# Autodesk Inventor assembly: LEG2
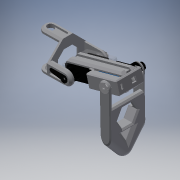
[picture p0: Inventor's stored thumbnail of the model, 180x180]
Saved by Autodesk Inventor 2017 (Build 210142000, 142)
## iProperties
Created: 2017-09-24
Part Number: LEG2
Document SubType Name: Assembly
Designer: Alexander Miller
Author: Alexander Miller
## Documents named in this file (12)
- X:\Alex\Documents\Git\HeRo-Mini\Hardware\LEG.iam
- X:\Alex\Documents\Git\HeRo-Mini\Hardware\SERVO.iam
- X:\Alex\Documents\Git\HeRo-Mini\Hardware\COXA.ipt
- X:\Alex\Documents\Git\HeRo-Mini\Hardware\FEMUR_A.ipt
- X:\Alex\Documents\Git\HeRo-Mini\Hardware\FEMUR_B.ipt
- X:\Alex\Documents\Git\HeRo-Mini\Hardware\BEARING.ipt
- X:\Alex\Documents\Git\HeRo-Mini\Hardware\TIBIA.ipt
- X:\Alex\Documents\Git\HeRo-Mini\Hardware\NUT_3MM.ipt
- X:\Alex\Documents\Git\HeRo-Mini\Hardware\NUT_2MM.ipt
- X:\Alex\Documents\Git\HeRo-Mini\Hardware\M2_SCREW_8MM.ipt
- X:\Alex\Documents\Git\HeRo-Mini\Hardware\M3_WASHER.ipt
- X:\Alex\Documents\Git\HeRo-Mini\Hardware\M3_SCREW_8MM.ipt
## Components (23 placed, 11 different names)
1. SERVO:1 [sub-assembly] — Rigid:1, Rigid:3, Rigid:7
2. SERVO:2 [sub-assembly] — Rigid:2, Rigid:4, Rigid:6
3. COXA:1 — Rotational:1, Rotational:2, Rigid:7
4. FEMUR_A:1 — Rigid:1, Rigid:2, Rigid:10, Rigid:11, Rigid:12, Rigid:13
5. FEMUR_B:1 — Rigid:4, Rigid:8, Rigid:15, Rigid:17
6. FEMUR_B:2 — Rigid:3, Rigid:9, Rigid:14, Rigid:16
7. BEARING:1 — Rotational:1, Rigid:18, Rotational:4
8. BEARING:2 — Rotational:2
9. TIBIA:1 — Rotational:3, Rigid:6
10. BEARING:3 — Rotational:3
11. NUT_3MM:1 — Rigid:9
12. NUT_3MM:2 — Rigid:8
13. NUT_2MM:1 — Rigid:10
14. NUT_2MM:2 — Rigid:11
15. NUT_2MM:3 — Rigid:12
16. NUT_2MM:4 — Rigid:13
17. M2_SCREW_8MM:1 — Rigid:14
18. M2_SCREW_8MM:2 — Rigid:15
19. M2_SCREW_8MM:3 — Rigid:16
20. M2_SCREW_8MM:4 — Rigid:17
21. M3_WASHER:1 — Rigid:18, Rigid:19
22. M3_WASHER:2 — Rigid:19
23. M3_SCREW_8MM:1 — Rotational:4
## Relationships (22: WeldJoint 18, RevoluteJoint 4)
- Rigid:1 [WeldJoint]: SERVO:1 ↔ FEMUR_A:1
- Rigid:2 [WeldJoint]: SERVO:2 ↔ FEMUR_A:1
- Rigid:3 [WeldJoint]: SERVO:1 ↔ FEMUR_B:2
- Rigid:4 [WeldJoint]: SERVO:2 ↔ FEMUR_B:1
- Rotational:1 [RevoluteJoint]: COXA:1 ↔ BEARING:1
- Rotational:2 [RevoluteJoint]: COXA:1 ↔ BEARING:2
- Rotational:3 [RevoluteJoint]: TIBIA:1 ↔ BEARING:3
- Rigid:6 [WeldJoint]: SERVO:2 ↔ TIBIA:1
- Rigid:7 [WeldJoint]: SERVO:1 ↔ COXA:1
- Rigid:8 [WeldJoint]: FEMUR_B:1 ↔ NUT_3MM:2
- Rigid:9 [WeldJoint]: FEMUR_B:2 ↔ NUT_3MM:1
- Rigid:10 [WeldJoint]: FEMUR_A:1 ↔ NUT_2MM:1
- Rigid:11 [WeldJoint]: FEMUR_A:1 ↔ NUT_2MM:2
- Rigid:12 [WeldJoint]: FEMUR_A:1 ↔ NUT_2MM:3
- Rigid:13 [WeldJoint]: FEMUR_A:1 ↔ NUT_2MM:4
- Rigid:14 [WeldJoint]: FEMUR_B:2 ↔ M2_SCREW_8MM:1
- Rigid:15 [WeldJoint]: FEMUR_B:1 ↔ M2_SCREW_8MM:2
- Rigid:16 [WeldJoint]: FEMUR_B:2 ↔ M2_SCREW_8MM:3
- Rigid:17 [WeldJoint]: FEMUR_B:1 ↔ M2_SCREW_8MM:4
- Rigid:18 [WeldJoint]: BEARING:1 ↔ M3_WASHER:1
- Rigid:19 [WeldJoint]: M3_WASHER:1 ↔ M3_WASHER:2
- Rotational:4 [RevoluteJoint]: BEARING:1 ↔ M3_SCREW_8MM:1
